# Autodesk Inventor assembly: Parqueo
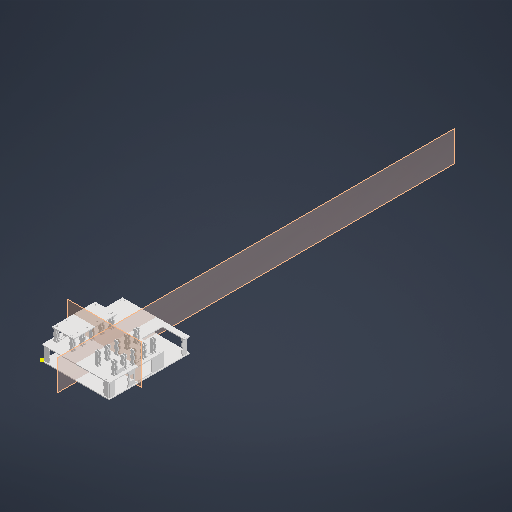
[picture p0: Inventor's stored thumbnail of the model, 512x512]
Saved by Autodesk Inventor 2026 (Build 300175000, 175)
## iProperties
Created: 2026-05-15
Part Number: Parqueo
Document SubType Name: Assembly
Designer: juana
Author: juana
## Documents named in this file (14)
- C:\Users\juana\OneDrive\Documentos\GitHub\Digital_2\ModuloSTM32\Nucleo1Paqueo\Modelo3DPark\Parqueo.iam
- C:\Users\juana\OneDrive\Documentos\GitHub\Digital_2\ModuloSTM32\Nucleo1Paqueo\Modelo3DPark\Base_de_equipo.ipt
- C:\Users\juana\OneDrive\Documentos\GitHub\Digital_2\ModuloSTM32\Nucleo1Paqueo\Modelo3DPark\soporte_base_parqueo.ipt
- C:\Users\juana\OneDrive\Documentos\GitHub\Digital_2\ModuloSTM32\Nucleo1Paqueo\Modelo3DPark\soporte_base_parqueo_MIR3.ipt
- C:\Users\juana\OneDrive\Documentos\GitHub\Digital_2\ModuloSTM32\Nucleo1Paqueo\Modelo3DPark\soporte_base_parqueo_MIR4.ipt
- C:\Users\juana\OneDrive\Documentos\GitHub\Digital_2\ModuloSTM32\Nucleo1Paqueo\Modelo3DPark\soporte_base_parqueo_MIR3_MIR.ipt
- C:\Users\juana\OneDrive\Documentos\GitHub\Digital_2\ModuloSTM32\Nucleo1Paqueo\Modelo3DPark\base_parqueo.ipt
- C:\Users\juana\OneDrive\Documentos\GitHub\Digital_2\ModuloSTM32\Nucleo1Paqueo\Modelo3DPark\columna_techo.ipt
- C:\Users\juana\OneDrive\Documentos\GitHub\Digital_2\ModuloSTM32\Nucleo1Paqueo\Modelo3DPark\columna_techo_MIR.ipt
- C:\Users\juana\OneDrive\Documentos\GitHub\Digital_2\ModuloSTM32\Nucleo1Paqueo\Modelo3DPark\columna2.ipt
- C:\Users\juana\OneDrive\Documentos\GitHub\Digital_2\ModuloSTM32\Nucleo1Paqueo\Modelo3DPark\techo.ipt
- C:\Users\juana\OneDrive\Documentos\GitHub\Digital_2\ModuloSTM32\Nucleo1Paqueo\Modelo3DPark\pantallaSoport.ipt
- C:\Users\juana\OneDrive\Documentos\GitHub\Digital_2\ModuloSTM32\Nucleo1Paqueo\Modelo3DPark\protector hal.ipt
- C:\Users\juana\OneDrive\Documentos\GitHub\Digital_2\ModuloSTM32\Nucleo1Paqueo\Modelo3DPark\techoProctetorSensorHal.ipt
## Components (56 placed, 13 different names)
1. Base_de_equipo:1 — Mate:2, Mate:3, Mate:4, Mate:5, Mate:6, Flush:1, Mate:7, Mate:8, Mate:9
2. base_parqueo:1 — Mate:10, Flush:2, Mate:11, Mate:12, Mate:13, Mate:14, Mate:15, Mate:16, Mate:17, Mate:19, Mate:24, Flush:4, Flush:5, Mate:26, Flush:28, Mate:28, Mate:29
3. columna2:1 — Mate:18, Mate:19, Mate:20
4. techo:1 — Mate:21, Mate:22, Mate:23
5. pantallaSoport:1 — Mate:25, Flush:6, Mate:26
6. soporte_base_parqueo:7 — Mate:24, Flush:4, Flush:5, Mate:25, Flush:6
7. protector hal:1 — Flush:28, Mate:28, Mate:29, Mate:30, Mate:31
8. techoProctetorSensorHal:1 — Mate:30, Mate:31
9. soporte_base_parqueo:1 — Mate:2, Mate:3, Mate:4
10. soporte_base_parqueo:6 — Mate:5, Mate:6, Flush:1
11. soporte_base_parqueo_MIR3:1 — Mate:10, Flush:2, Mate:11
12. soporte_base_parqueo_MIR3:2
13. soporte_base_parqueo_MIR4:1
14. soporte_base_parqueo_MIR4:2
15. soporte_base_parqueo_MIR3_MIR:1
16. soporte_base_parqueo_MIR3_MIR:2
17. columna_techo:2 — Mate:15, Mate:16, Mate:17, Mate:18, Mate:20, Mate:23
18. columna_techo:1 — Mate:12, Mate:13, Mate:14
19. columna_techo:3
20. columna_techo:4
21. columna_techo:5
22. columna_techo:6
23. columna_techo:7
24. columna_techo:8
25. columna_techo:9
26. columna_techo:10
27. columna_techo:11
28. columna_techo:12
29. columna_techo:13
30. columna_techo:14
31. columna_techo:15
32. columna_techo:16
33. columna_techo:17 — Mate:22
34. columna_techo:18 — Mate:21
35. columna_techo:19
36. columna_techo:20
37. columna_techo_MIR:2
38. columna_techo_MIR:1
39. columna_techo_MIR:3
40. columna_techo_MIR:4
41. columna_techo_MIR:5
42. columna_techo_MIR:6
43. columna_techo_MIR:7
44. columna_techo_MIR:8
45. columna_techo_MIR:9
46. columna_techo_MIR:10
47. columna_techo_MIR:11
48. columna_techo_MIR:12
49. columna_techo_MIR:13
50. columna_techo_MIR:14
51. columna_techo_MIR:15
52. columna_techo_MIR:16
53. columna_techo_MIR:17
54. columna_techo_MIR:18
55. columna_techo_MIR:19
56. columna_techo_MIR:20
## Component patterns: (2 elements), (2 elements), (2 elements, first: soporte_base_parqueo:1 + soporte_base_parqueo:6), Mirror Component Pattern 4:2 (2 elements), (10 elements, first: columna_techo:2 + columna_techo:1), Component Pattern 6:2 (10 elements)
## Relationships (36: Mate 29, Flush 7)
- Mate:2: Base_de_equipo:1 ↔ soporte_base_parqueo:1
- Mate:3: Base_de_equipo:1 ↔ soporte_base_parqueo:1
- Mate:4: Base_de_equipo:1 ↔ soporte_base_parqueo:1
- Mate:5: Base_de_equipo:1 ↔ soporte_base_parqueo:6
- Mate:6: Base_de_equipo:1 ↔ soporte_base_parqueo:6
- Flush:1: Base_de_equipo:1 ↔ soporte_base_parqueo:6
- Mate:7: Base_de_equipo:1
- Mate:8: Base_de_equipo:1
- Mate:9: Base_de_equipo:1
- Mate:10: base_parqueo:1 ↔ soporte_base_parqueo_MIR3:1
- Flush:2: base_parqueo:1 ↔ soporte_base_parqueo_MIR3:1
- Mate:11: base_parqueo:1 ↔ soporte_base_parqueo_MIR3:1
- Mate:12: base_parqueo:1 ↔ columna_techo:1
- Mate:13: base_parqueo:1 ↔ columna_techo:1
- Mate:14: base_parqueo:1 ↔ columna_techo:1
- Flush:3 (41.5 mm)
- Mate:15: base_parqueo:1 ↔ columna_techo:2
- Mate:16: base_parqueo:1 ↔ columna_techo:2
- Mate:17: base_parqueo:1 ↔ columna_techo:2
- Mate:18: columna2:1 ↔ columna_techo:2
- Mate:19: base_parqueo:1 ↔ columna2:1
- Mate:20: columna2:1 ↔ columna_techo:2
- Mate:21: techo:1 ↔ columna_techo:18
- Mate:22: techo:1 ↔ columna_techo:17
- Mate:23: techo:1 ↔ columna_techo:2
- Mate:24: base_parqueo:1 ↔ soporte_base_parqueo:7
- Flush:4: base_parqueo:1 ↔ soporte_base_parqueo:7
- Flush:5: base_parqueo:1 ↔ soporte_base_parqueo:7
- Mate:25: pantallaSoport:1 ↔ soporte_base_parqueo:7
- Flush:6: pantallaSoport:1 ↔ soporte_base_parqueo:7
- Mate:26: base_parqueo:1 ↔ pantallaSoport:1
- Flush:28: base_parqueo:1 ↔ protector hal:1
- Mate:28: base_parqueo:1 ↔ protector hal:1
- Mate:29: base_parqueo:1 ↔ protector hal:1
- Mate:30: protector hal:1 ↔ techoProctetorSensorHal:1
- Mate:31: protector hal:1 ↔ techoProctetorSensorHal:1
